# Autodesk Inventor assembly: ASY PNS 00 Panaevsk VOS
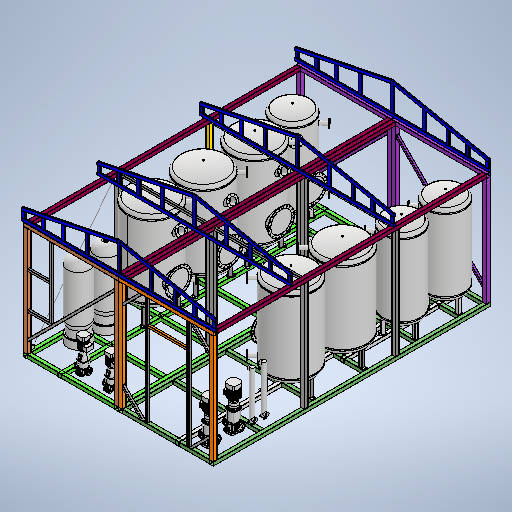
[picture p0: Inventor's stored thumbnail of the model, 512x512]
Saved by Autodesk Inventor 2025.1 (Build 291241020, 241B)
## iProperties
Created: 2025-02-24
Part Number: ASY PNS 00 Panaevsk VOS
Document SubType Name: Assembly
Designer: user
Author: user
## Documents named in this file (14)
- C:\Users\user\YandexDisk-badmisterfox\home pc\Inventor\PNS-Panaevsk\ASY PNS 00 Panaevsk VOS.iam
- C:\Users\user\YandexDisk-badmisterfox\home pc\Inventor\PNS-Panaevsk\D1000\ASY PNS-Filter column D1200.iam
- C:\Users\user\YandexDisk-badmisterfox\home pc\Inventor\PNS-Panaevsk\Filter D1200\ASY PNS-Filter column D1000.iam
- C:\Users\user\YandexDisk-badmisterfox\home pc\Inventor\PNS-Panaevsk\ASY PNS-0100 MAIN FRAME.iam
- C:\Users\user\YandexDisk-badmisterfox\home pc\Inventor\PNS-Panaevsk\ASY PNS-0200 FRAME 2.ipt
- C:\Users\user\YandexDisk-badmisterfox\home pc\Inventor\PNS-Panaevsk\PNS-0410 filter pillar.ipt
- C:\Users\user\YandexDisk-badmisterfox\home pc\Inventor\PNS-Panaevsk\PNS-0921 concrete plate.ipt
- C:\Users\user\YandexDisk-badmisterfox\home pc\Inventor\PNS-Panaevsk\PNS-0931 Sandwich wall.ipt
- C:\Users\user\YandexDisk-badmisterfox\home pc\Inventor\PNS-Panaevsk\PNS-0932 Sandwich wall roof.ipt
- C:\Users\user\YandexDisk-badmisterfox\home pc\Inventor\PNS-Panaevsk\PNS-0264 roof beam.ipt
- C:\Users\user\YandexDisk-badmisterfox\home pc\Inventor\PNS-Panaevsk\Оборудование Инвентор\Вертикальный насос\CDM(F)15-4 FSWP(S_L)C\CDM(F)15-4 FSWP(S_L)C.iam
- C:\Users\user\YandexDisk-badmisterfox\home pc\Inventor\PNS-Panaevsk\Оборудование Инвентор\Вертикальный насос\CDM(F)65-2-2 FSWP(S)C\CDM(F)65-2-2 FSWP(S)C.iam
- C:\Users\user\YandexDisk-badmisterfox\home pc\Inventor\PNS-Panaevsk\Оборудование Инвентор\HY-H H2162–4T.ipt
- C:\Users\user\YandexDisk-badmisterfox\home pc\Inventor\PNS-Panaevsk\Оборудование Инвентор\UV-Cleaner ODV-15.ipt
## Components (29 placed, 13 different names)
1. ASY PNS-Filter column D1200:2 [sub-assembly] — Rigid:13
2. ASY PNS-Filter column D1000:3 [sub-assembly] — Rigid:6
3. ASY PNS-Filter column D1000:5 [sub-assembly] — Rigid:10
4. ASY PNS-0100 MAIN FRAME:1 [sub-assembly] — Rigid:1, Rigid:3, Rigid:4, Rigid:5, Rigid:6, Rigid:7, Rigid:8, Rigid:9, Rigid:10, Rigid:11, Rigid:12, Rigid:13, Mate:15, Mate:16, Mate:17, Mate:18, Mate:19, Mate:20, Mate:21, Mate:22
5. ASY PNS-0200 FRAME 2:1
6. PNS-0410 filter pillar:1
7. ASY PNS-Filter column D1200:5 [sub-assembly] — Rigid:12
8. ASY PNS-Filter column D1200:6 [sub-assembly] — Rigid:8
9. ASY PNS-Filter column D1200:7 [sub-assembly] — Rigid:9
10. PNS-0931 Sandwich wall:1 — Rigid:1
11. PNS-0932 Sandwich wall roof:1 — Rigid:2
12. PNS-0932 Sandwich wall roof:2 — Rigid:2
13. PNS-0264 roof beam:1 — Rigid:3
14. PNS-0264 roof beam:2 — Rigid:4
15. PNS-0264 roof beam:3 — Rigid:5
16. ASY PNS-Filter column D1200:8 [sub-assembly] — Rigid:7
17. ASY PNS-Filter column D1000:6 [sub-assembly] — Rigid:11
18. CDM(F)15-4 FSWP(S_L)C:1 [sub-assembly] — Mate:16
19. CDM(F)65-2-2 FSWP(S)C:1 [sub-assembly] — Mate:18
20. HY-H H2162–4T:1 — Mate:19
21. UV-Cleaner ODV-15:1 — Mate:22
22. UV-Cleaner ODV-15:2 — Mate:21
23. HY-H H2162–4T:2 — Mate:20
24. CDM(F)65-2-2 FSWP(S)C:2 [sub-assembly] — Mate:17
25. CDM(F)15-4 FSWP(S_L)C:2 [sub-assembly] — Mate:15
26. PNS-0921 concrete plate:1 — Flush:6, Flush:7, Mate:14
27. PNS-0921 concrete plate:2
28. PNS-0921 concrete plate:3
29. PNS-0921 concrete plate:4
## Component patterns: (4 elements, first: PNS-0921 concrete plate:1)
## Relationships (24: WeldJoint 13, Mate 9, Flush 2)
- Flush:6: PNS-0921 concrete plate:1
- Flush:7: PNS-0921 concrete plate:1
- Mate:14 (-500 mm): PNS-0921 concrete plate:1
- Rigid:1 [WeldJoint]: ASY PNS-0100 MAIN FRAME:1 ↔ PNS-0931 Sandwich wall:1
- Rigid:2 [WeldJoint]: PNS-0932 Sandwich wall roof:1 ↔ PNS-0932 Sandwich wall roof:2
- Rigid:3 [WeldJoint]: ASY PNS-0100 MAIN FRAME:1 ↔ PNS-0264 roof beam:1
- Rigid:4 [WeldJoint]: ASY PNS-0100 MAIN FRAME:1 ↔ PNS-0264 roof beam:2
- Rigid:5 [WeldJoint]: ASY PNS-0100 MAIN FRAME:1 ↔ PNS-0264 roof beam:3
- Rigid:6 [WeldJoint]: ASY PNS-Filter column D1000:3 ↔ ASY PNS-0100 MAIN FRAME:1
- Rigid:7 [WeldJoint]: ASY PNS-0100 MAIN FRAME:1 ↔ ASY PNS-Filter column D1200:8
- Rigid:8 [WeldJoint]: ASY PNS-0100 MAIN FRAME:1 ↔ ASY PNS-Filter column D1200:6
- Rigid:9 [WeldJoint]: ASY PNS-0100 MAIN FRAME:1 ↔ ASY PNS-Filter column D1200:7
- Rigid:10 [WeldJoint]: ASY PNS-Filter column D1000:5 ↔ ASY PNS-0100 MAIN FRAME:1
- Rigid:11 [WeldJoint]: ASY PNS-0100 MAIN FRAME:1 ↔ ASY PNS-Filter column D1000:6
- Rigid:12 [WeldJoint]: ASY PNS-0100 MAIN FRAME:1 ↔ ASY PNS-Filter column D1200:5
- Rigid:13 [WeldJoint]: ASY PNS-Filter column D1200:2 ↔ ASY PNS-0100 MAIN FRAME:1
- Mate:15: ASY PNS-0100 MAIN FRAME:1 ↔ CDM(F)15-4 FSWP(S_L)C:2
- Mate:16: ASY PNS-0100 MAIN FRAME:1 ↔ CDM(F)15-4 FSWP(S_L)C:1
- Mate:17: ASY PNS-0100 MAIN FRAME:1 ↔ CDM(F)65-2-2 FSWP(S)C:2
- Mate:18: ASY PNS-0100 MAIN FRAME:1 ↔ CDM(F)65-2-2 FSWP(S)C:1
- Mate:19: ASY PNS-0100 MAIN FRAME:1 ↔ HY-H H2162–4T:1
- Mate:20: ASY PNS-0100 MAIN FRAME:1 ↔ HY-H H2162–4T:2
- Mate:21: ASY PNS-0100 MAIN FRAME:1 ↔ UV-Cleaner ODV-15:2
- Mate:22: ASY PNS-0100 MAIN FRAME:1 ↔ UV-Cleaner ODV-15:1
